# Autodesk Inventor assembly: Lamp
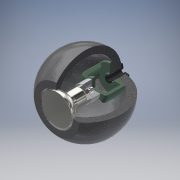
[picture p0: Inventor's stored thumbnail of the model, 180x180]
Saved by Autodesk Inventor 2018.2 (Build 222227000, 227)
## iProperties
Created: 2018-01-26
Part Number: Lamp
Material: Generisch
Document SubType Name: Assembly
Designer: JochenAlt
Author: JochenAlt
## Documents named in this file (8)
- D:\Projects\concretelamp\CAD\Sphere\Lamp.iam
- D:\Projects\concretelamp\CAD\Sphere\CableStrainRelief.ipt
- D:\Projects\concretelamp\CAD\Sphere\Inlet.ipt
- D:\Projects\concretelamp\CAD\Sphere\Lamp.ipt
- D:\Projects\concretelamp\CAD\GU10-Socket.ipt
- C:\Users\JochenAlt\Documents\Inventor\Content Center Files\R2018\de-DE\DIN 912\DIN 912 - M3 x 0,5 x 12 x 10,75.ipt
- C:\Users\JochenAlt\Documents\Inventor\Content Center Files\R2018\de-DE\AS 1112 (2)\AS 1112 - M3  Typ 8.ipt
- D:\Projects\concretelamp\CAD\Bulb GU10\Bulb GU10.iam
## Components (9 placed, 7 different names)
1. Cable Strain Relief:1 — Passend:38, Passend:39, Passend:40, Fluchtend:1
2. Inlet:1 — Passend:25, Passend:26, Passend:29, Passend:35, Passend:37, Passend:40, Fluchtend:1
3. Lamp:1 — Passend:38, Passend:39, Passend:41, Fluchtend:2
4. GU10-Socket:1 — Passend:25, Passend:26, Passend:29, Passend:30, Passend:31, Passend:32, Passend:33
5. DIN 912 - ersetzt durch DIN EN ISO 4762 M3 x 12:1 — Passend:30, Passend:31, Passend:34
6. DIN 912 - ersetzt durch DIN EN ISO 4762 M3 x 12:2 — Passend:32, Passend:33, Passend:36
7. AS 1112 (2) - Metrisch M3  Typ 8:1 — Passend:34, Passend:35
8. AS 1112 (2) - Metrisch M3  Typ 8:2 — Passend:36, Passend:37
9. Bulb GU10:1 [sub-assembly] — Passend:41, Fluchtend:2
## Relationships (17: Mate 15, Flush 2)
- Passend:25 [Mate]: Inlet:1 ↔ GU10-Socket:1
- Passend:26 [Mate] (0.3 mm): Inlet:1 ↔ GU10-Socket:1
- Passend:29 [Mate]: Inlet:1 ↔ GU10-Socket:1
- Passend:30 [Mate]: GU10-Socket:1 ↔ DIN 912 - ersetzt durch DIN EN ISO 4762 M3 x 12:1
- Passend:31 [Mate]: GU10-Socket:1 ↔ DIN 912 - ersetzt durch DIN EN ISO 4762 M3 x 12:1
- Passend:32 [Mate]: GU10-Socket:1 ↔ DIN 912 - ersetzt durch DIN EN ISO 4762 M3 x 12:2
- Passend:33 [Mate]: GU10-Socket:1 ↔ DIN 912 - ersetzt durch DIN EN ISO 4762 M3 x 12:2
- Passend:34 [Mate]: DIN 912 - ersetzt durch DIN EN ISO 4762 M3 x 12:1 ↔ AS 1112 (2) - Metrisch M3  Typ 8:1
- Passend:35 [Mate]: Inlet:1 ↔ AS 1112 (2) - Metrisch M3  Typ 8:1
- Passend:36 [Mate]: DIN 912 - ersetzt durch DIN EN ISO 4762 M3 x 12:2 ↔ AS 1112 (2) - Metrisch M3  Typ 8:2
- Passend:37 [Mate]: Inlet:1 ↔ AS 1112 (2) - Metrisch M3  Typ 8:2
- Passend:38 [Mate]: Cable Strain Relief:1 ↔ Lamp:1
- Passend:39 [Mate]: Cable Strain Relief:1 ↔ Lamp:1
- Passend:40 [Mate]: Cable Strain Relief:1 ↔ Inlet:1
- Fluchtend:1 [Flush] (0.4 mm): Cable Strain Relief:1 ↔ Inlet:1
- Passend:41 [Mate]: Lamp:1 ↔ Bulb GU10:1
- Fluchtend:2 [Flush]: Lamp:1 ↔ Bulb GU10:1
